# Autodesk Inventor assembly: WheelStrutLocomotion
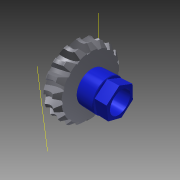
[picture p0: Inventor's stored thumbnail of the model, 180x180]
Saved by Autodesk Inventor 2014 (Build 180170000, 170)
## iProperties
Created: 2014-08-24
Part Number: WheelStrutLocomotion
Document SubType Name: Assembly
Designer: sam
Author: sam
## Documents named in this file (8)
- C:\Users\sam\Desktop\Octanis-CAD-Windows\WheelStrutLocomotion.iam
- C:\Users\sam\Desktop\Octanis-CAD-Windows\WheelStrutLocomotion\Design Accelerator\Shaft1.iam
- C:\Users\sam\Desktop\Octanis-CAD-Windows\WheelStrutLocomotion\Design Accelerator\Shaft3.iam
- C:\Users\sam\Desktop\Octanis-CAD-Windows\WheelStrutLocomotion\Design Accelerator\Worm Gears2.iam
- C:\Users\sam\Desktop\Octanis-CAD-Windows\WheelStrutLocomotion\Design Accelerator\Worm Gears4.iam
- C:\Users\sam\Desktop\Octanis-CAD-Windows\WheelStrutLocomotion\Design Accelerator\Worm Gears5.iam
- C:\Users\sam\Desktop\Octanis-CAD-Windows\WheelStrutLocomotion\Design Accelerator\Shaft4.iam
- C:\Users\sam\Desktop\Octanis-CAD-Windows\WheelStrutLocomotion\Design Accelerator\Shaft5.iam
## Components (6 placed, 2 different names)
1. Shaft:1 [sub-assembly] — Insert:3, Cylindrical:1
2. Shaft:2 [sub-assembly] — Cylindrical:1, Mate:8, Mate:9, Insert:4, Mate:10, Angle:1
3. Worm Gears:3 [sub-assembly] — Insert:3, Mate:11, Mate:16, Angle:2
4. Worm Gears:4 [sub-assembly] — Insert:4, Mate:10, Mate:12, Mate:14
5. Shaft:3 [sub-assembly] — Mate:13, Mate:14, Angle:1
6. Shaft:4 [sub-assembly] — Mate:15, Mate:16, Angle:2
## Relationships (14: Mate 9, Insert 2, Angle 2, CylindricalJoint 1)
- Insert:3: Shaft:1 ↔ Worm Gears:3
- Cylindrical:1: Shaft:1 ↔ Shaft:2
- Mate:8: Shaft:2
- Mate:9: Shaft:2
- Insert:4: Shaft:2 ↔ Worm Gears:4
- Mate:10: Shaft:2 ↔ Worm Gears:4
- Mate:11: Worm Gears:3
- Mate:12: Worm Gears:4
- Mate:13: Shaft:3
- Mate:14 (5.8208 mm): Worm Gears:4 ↔ Shaft:3
- Angle:1 (0 deg): Shaft:2 ↔ Shaft:3
- Mate:15: Shaft:4
- Mate:16 (6 mm): Worm Gears:3 ↔ Shaft:4
- Angle:2 (0 deg): Worm Gears:3 ↔ Shaft:4
